# Autodesk Inventor assembly: HubBoltWithLockNut
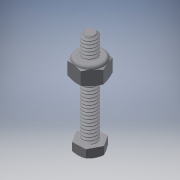
[picture p0: Inventor's stored thumbnail of the model, 180x180]
Saved by Autodesk Inventor 2016 (Build 200138000, 138)
## iProperties
Created: 2017-01-08
Part Number: HubBoltWithLockNut
Document SubType Name: Assembly
Designer: Dhruv
Author: Dhruv
## Documents named in this file (3)
- C:\Users\Dhruv\Desktop\MISC\FRC 2017\HubBoltWithLockNut.iam
- C:\Users\Dhruv\Desktop\MISC\FRC 2017\supporting_parts\93075A249_ZINC-PLATED STEEL HEX HEAD MACHINE SCREW.ipt
- C:\Users\Dhruv\Desktop\MISC\FRC 2017\supporting_parts\90631A011_LOW-STRENGTH STEEL NYLON-INSERT LOCKNUT.ipt
## Components (2 placed, 2 different names)
1. 93075A249_ZINC-PLATED STEEL HEX HEAD MACHINE SCREW:1
2. 90631A011_LOW-STRENGTH STEEL NYLON-INSERT LOCKNUT:1
## Relationships (1: Mate 1)
- [Mate]: 93075A249_ZINC-PLATED STEEL HEX HEAD MACHINE SCREW:1 ↔ 90631A011_LOW-STRENGTH STEEL NYLON-INSERT LOCKNUT:1
